# Autodesk Inventor assembly: NPTC102KFMS-RC
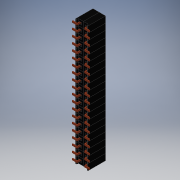
[picture p0: Inventor's stored thumbnail of the model, 180x180]
Saved by Autodesk Inventor 2016 (Build 200138000, 138)
## iProperties
Created: 2016-08-01
Part Number: NPTC102KFMS-RC
Document SubType Name: Assembly
Designer: Jonathan
Author: Jonathan
## Documents named in this file (3)
- C:\Users\Jonathan\Documents\Projects\mppcInterface\4-channel\mppcInterface\cad\connector\NPTC102KFMS-RC\NPTC102KFMS-RC.iam
- C:\Users\Jonathan\Documents\Projects\mppcInterface\4-channel\mppcInterface\cad\connector\NPTC102KFMS-RC\body.ipt
- C:\Users\Jonathan\Documents\Projects\mppcInterface\4-channel\mppcInterface\cad\connector\NPTC102KFMS-RC\pin.ipt
## Components (160 placed, 2 different names)
1. pin:1 — Mate:1, Mate:2, Flush:1
2. body:1 — Mate:1, Mate:2, Flush:1
3. pin:2
4. body:2
5. pin:3
6. body:3
7. pin:4
8. body:4
9. pin:5
10. body:5
11. pin:6
12. body:6
13. pin:7
14. body:7
15. pin:8
16. body:8
17. pin:9
18. body:9
19. pin:10
20. body:10
21. pin:11
22. body:11
23. pin:12
24. body:12
25. pin:13
26. body:13
27. pin:14
28. body:14
29. pin:15
30. body:15
31. pin:16
32. body:16
33. pin:17
34. body:17
35. pin:18
36. body:18
37. pin:19
38. body:19
39. pin:20
40. body:20
41. pin:21
42. body:21
43. pin:22
44. body:22
45. pin:23
46. body:23
47. pin:24
48. body:24
49. pin:25
50. body:25
51. pin:26
52. body:26
53. pin:27
54. body:27
55. pin:28
56. body:28
57. pin:29
58. body:29
59. pin:30
60. body:30
61. pin:31
62. body:31
63. pin:32
64. body:32
65. pin:33
66. body:33
67. pin:34
68. body:34
69. pin:35
70. body:35
71. pin:36
72. body:36
73. pin:37
74. body:37
75. pin:38
76. body:38
77. pin:39
78. body:39
79. pin:40
80. body:40
81. pin:41
82. body:41
83. pin:42
84. body:42
85. pin:43
86. body:43
87. pin:44
88. body:44
89. pin:45
90. body:45
91. pin:46
92. body:46
93. pin:47
94. body:47
95. pin:48
96. body:48
97. pin:49
98. body:49
99. pin:50
100. body:50
101. pin:51
102. body:51
103. pin:52
104. body:52
105. pin:53
106. body:53
107. pin:54
108. body:54
109. pin:55
110. body:55
111. pin:56
112. body:56
113. pin:57
114. body:57
115. pin:58
116. body:58
117. pin:59
118. body:59
119. pin:60
120. body:60
121. pin:61
122. body:61
123. pin:62
124. body:62
125. pin:63
126. body:63
127. pin:64
128. body:64
129. pin:65
130. body:65
131. pin:66
132. body:66
133. pin:67
134. body:67
135. pin:68
136. body:68
137. pin:69
138. body:69
139. pin:70
140. body:70
141. pin:71
142. body:71
143. pin:72
144. body:72
145. pin:73
146. body:73
147. pin:74
148. body:74
149. pin:75
150. body:75
151. pin:76
152. body:76
153. pin:77
154. body:77
155. pin:78
156. body:78
157. pin:79
158. body:79
159. pin:80
160. body:80
## Component patterns: (4 elements), (20 elements, first: pin:1 + body:1), Component Pattern 1:2 (20 elements), Component Pattern 1:3 (20 elements), Component Pattern 1:4 (20 elements)
## Relationships (3: Mate 2, Flush 1)
- Mate:1: pin:1 ↔ body:1
- Mate:2 (0.1346 mm): pin:1 ↔ body:1
- Flush:1: pin:1 ↔ body:1
